# Autodesk Inventor assembly: pulleyBracketAssembly
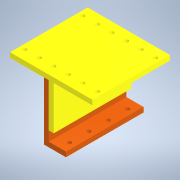
[picture p0: Inventor's stored thumbnail of the model, 180x180]
Saved by Autodesk Inventor 2022.1 (Build 261234020, 234B)
## iProperties
Created: 2021-11-11
Part Number: pulleyBracketAssembly
Document SubType Name: Assembly
Designer: robst
Author: robst
## Documents named in this file (3)
- C:\git\CAD-Development\robSteele\pulleyBracketAssembly.iam
- C:\git\CAD-Development\robSteele\pullyBracketLowerPortion.ipt
- C:\git\CAD-Development\robSteele\pullyBracketTopPortion.ipt
## Components (2 placed, 2 different names)
1. pullyBracketLowerPortion:1 — Mate:1, Flush:1, Mate:2
2. pullyBracketTopPortion:1 — Mate:1, Flush:1, Mate:2
## Relationships (3: Mate 2, Flush 1)
- Mate:1: pullyBracketLowerPortion:1 ↔ pullyBracketTopPortion:1
- Flush:1: pullyBracketLowerPortion:1 ↔ pullyBracketTopPortion:1
- Mate:2: pullyBracketLowerPortion:1 ↔ pullyBracketTopPortion:1
